# Autodesk Inventor assembly: PumpConcept
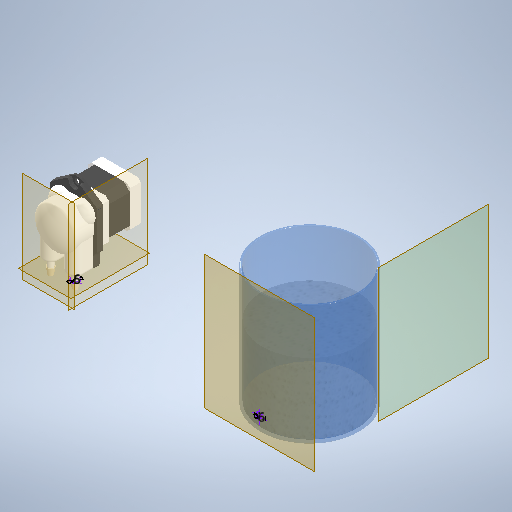
[picture p0: Inventor's stored thumbnail of the model, 512x512]
Saved by Autodesk Inventor 2025.2 (Build 292293000, 293)
## iProperties
Created: 2025-05-29
Part Number: PumpConcept
Document SubType Name: Assembly
Designer: Simon
Author: Simon
## Documents named in this file (4)
- C:\Users\Simon\OneDrive\Documents\Inventor\Skripsie2025\Extruder Concept 3\PumpConcept.iam
- C:\Users\Simon\OneDrive\Documents\Inventor\Skripsie2025\PartsFolder\Peristaltic Pump\Peristaltic Pump Assembly.iam
- C:\Users\Simon\OneDrive\Documents\Inventor\Skripsie2025\Extruder Concept 3\Gel.ipt
- C:\Users\Simon\OneDrive\Documents\Inventor\Skripsie2025\Extruder Concept 3\Reservoir.ipt
## Components (3 placed, 3 different names)
1. Peristaltic Pump Assembly:1 [sub-assembly] — Mate:1, Mate:2, Mate:3, Flush:1, Mate:7, Angle:1, Angle:3, Tangent:2
2. Gel:1 — Mate:4, Mate:5
3. Reservoir:1 — Mate:4, Mate:5, Mate:6, Tangent:1, Flush:2, Flush:3
## Relationships (16: Mate 8, Flush 3, Angle 3, Tangent 2)
- Mate:1: Peristaltic Pump Assembly:1
- Mate:2: Peristaltic Pump Assembly:1
- Mate:3: Peristaltic Pump Assembly:1
- Mate:4: Gel:1 ↔ Reservoir:1
- Mate:5: Gel:1 ↔ Reservoir:1
- Mate:6 (-40 mm): Reservoir:1
- Flush:1: Peristaltic Pump Assembly:1
- Mate:7: Peristaltic Pump Assembly:1
- Angle:1 (0 deg): Peristaltic Pump Assembly:1
- Angle:2 (0 deg)
- Tangent:1: Reservoir:1
- Mate:8 (200 mm)
- Angle:3 (0 deg): Peristaltic Pump Assembly:1
- Tangent:2: Peristaltic Pump Assembly:1
- Flush:2: Reservoir:1
- Flush:3: Reservoir:1
